# Autodesk Inventor assembly: 0011-Marco_apm_002-1
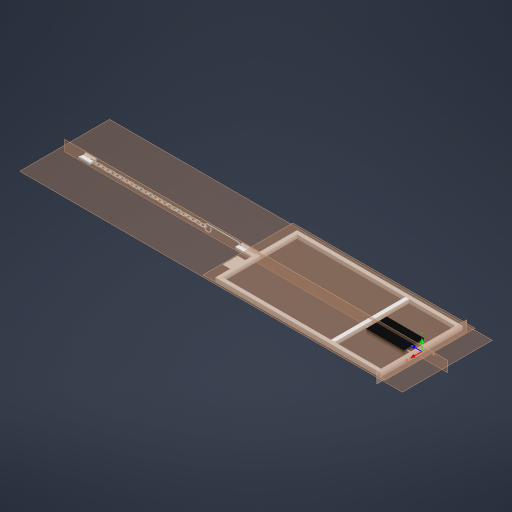
[picture p0: Inventor's stored thumbnail of the model, 512x512]
Saved by Autodesk Inventor 2024 (Build 280153000, 153)
## iProperties
Created: 2023-05-17
Part Number: 0011-Marco_apm_002-1
Document SubType Name: Assembly
Designer: javie
Author: javie
## Documents named in this file (8)
- C:\Users\javie\Downloads\Piezas CMR\S_RobotStudio_Model\0011-Marco_apm_002-1.iam
- C:\Users\javie\Downloads\Piezas CMR\Marco_Conveyor_Aereo.iam
- C:\Users\javie\Downloads\Piezas CMR\Marco_APM_002\Piezas\APM_002-1.ipt
- C:\Users\javie\Downloads\Piezas CMR\Marcos_solids\Pieza1.ipt
- C:\Users\javie\Downloads\Piezas CMR\S_RobotStudio_Model\Pieza2.ipt
- C:\Users\javie\Downloads\Piezas CMR\Marcos_solids\Topes_apm_002-2.ipt
- C:\Users\javie\Downloads\Piezas CMR\Marcos_solids\S_horizontal.ipt
- C:\Users\javie\Downloads\Piezas CMR\Marcos_solids\0011.ipt
## Components (7 placed, 7 different names)
1. Marco_Conveyor_Aereo:1 [sub-assembly] — Nivelación:1, Nivelación:3, Nivelación:4
2. APM_002-1:1 — Insertar:1, Nivelación:2, Insertar:2
3. Pieza1:1 — Nivelación:1, Insertar:1
4. Pieza2:1 — Nivelación:2
5. Topes_apm_002-2:1 — Insertar:2, Insertar:3
6. S_horizontal:1 — Insertar:3
7. 0011:1 — Nivelación:3, Nivelación:4
## Relationships (7: Flush 4, Insert 3)
- Nivelación:1 [Flush]: Marco_Conveyor_Aereo:1 ↔ Pieza1:1
- Insertar:1: APM_002-1:1 ↔ Pieza1:1
- Nivelación:2 [Flush]: APM_002-1:1 ↔ Pieza2:1
- Insertar:2: APM_002-1:1 ↔ Topes_apm_002-2:1
- Insertar:3: Topes_apm_002-2:1 ↔ S_horizontal:1
- Nivelación:3 [Flush]: Marco_Conveyor_Aereo:1 ↔ 0011:1
- Nivelación:4 [Flush]: Marco_Conveyor_Aereo:1 ↔ 0011:1
